# Autodesk Inventor assembly: Ensamble inicial_ Dog Feeder
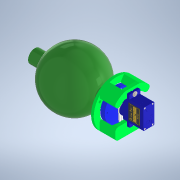
[picture p0: Inventor's stored thumbnail of the model, 180x180]
Saved by Autodesk Inventor 2020.1 (Build 241239000, 239)
## iProperties
Created: 2019-11-16
Part Number: Ensamble inicial_ Dog Feeder
Document SubType Name: Assembly
Designer: Daniel
Author: Daniel
## Documents named in this file (6)
- F:\Proyectos\Dog Feeder\Solido\Ensamble Inicial\Ensamble inicial_ Dog Feeder.iam
- F:\Proyectos\Dog Feeder\Solido\Ensamble Inicial\Dosificador.ipt
- F:\Proyectos\Dog Feeder\Solido\Ensamble Inicial\Exagono.ipt
- F:\Proyectos\Dog Feeder\Solido\Ensamble Inicial\Soporte_Servo.ipt
- F:\Proyectos\Dog Feeder\Solido\Servo SG90\SG90 - Micro Servo 9g - Tower Pro.iam
- C:\Users\Daniel\Documents\Inventor\Content Center Files\R2020\en-US\ISO 4762(2)\ISO 4762 - M1.6 x 8ISO.ipt
## Components (6 placed, 5 different names)
1. Dosificador:1
2. Exagono:1 — Insert:1, Mate:8, Rotational:1
3. Soporte_Servo:1 — Insert:2
4. SG90 - Micro Servo 9g - Tower Pro:1 [sub-assembly] — Insert:1, Mate:8, Flush:8, Insert:2
5. ISO 4762 M1.6 x 8:1 — Rotational:1
6. ISO 4762 M1.6 x 8:2
## Component patterns: (2 elements, first: ISO 4762 M1.6 x 8:1)
## Relationships (5: Insert 2, Mate 1, Flush 1, RevoluteJoint 1)
- Insert:1: Exagono:1 ↔ SG90 - Micro Servo 9g - Tower Pro:1
- Mate:8: Exagono:1 ↔ SG90 - Micro Servo 9g - Tower Pro:1
- Flush:8 (7.08 mm): SG90 - Micro Servo 9g - Tower Pro:1
- Rotational:1 [RevoluteJoint]: Exagono:1 ↔ ISO 4762 M1.6 x 8:1
- Insert:2: Soporte_Servo:1 ↔ SG90 - Micro Servo 9g - Tower Pro:1
